# Autodesk Inventor assembly: assembly
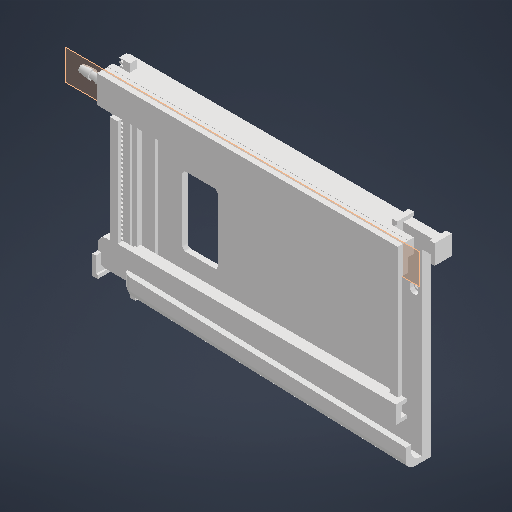
[picture p0: Inventor's stored thumbnail of the model, 512x512]
Saved by Autodesk Inventor 2026.2 (Build 302298010, 298A)
## iProperties
Created: 2026-07-05
Part Number: assembly
Document SubType Name: Assembly
Designer: pauli
Author: pauli
## Documents named in this file (6)
- D:\Documentos\auto-cleaning-solar-panel\hardware\CAD\iam\assembly.iam
- D:\Documentos\auto-cleaning-solar-panel\hardware\CAD\ipt\Gear.ipt
- D:\Documentos\auto-cleaning-solar-panel\hardware\CAD\ipt\Gear-Rack.ipt
- D:\Documentos\auto-cleaning-solar-panel\hardware\CAD\ipt\panel-suport.ipt
- D:\Documentos\auto-cleaning-solar-panel\hardware\CAD\ipt\Sprinkler.ipt
- D:\Documentos\auto-cleaning-solar-panel\hardware\CAD\ipt\Wiper-support.ipt
## Components (5 placed, 5 different names)
1. Gear:1 — Coincidente:7, Alinhado:1, Coincidente:8
2. Gear-Rack:1 — Coincidente:4, Coincidente:5, Coincidente:6, Coincidente:7, Alinhado:1, Coincidente:8
3. panel-suport:1 — Coincidente:1, Coincidente:2, Coincidente:3, Coincidente:4, Coincidente:5
4. Sprinkler:1 — Coincidente:1, Coincidente:2, Coincidente:3
5. Wiper-support:1 — Coincidente:6
## Relationships (9: Mate 8, Flush 1)
- Coincidente:1 [Mate]: panel-suport:1 ↔ Sprinkler:1
- Coincidente:2 [Mate]: panel-suport:1 ↔ Sprinkler:1
- Coincidente:3 [Mate]: panel-suport:1 ↔ Sprinkler:1
- Coincidente:4 [Mate]: Gear-Rack:1 ↔ panel-suport:1
- Coincidente:5 [Mate]: Gear-Rack:1 ↔ panel-suport:1
- Coincidente:6 [Mate]: Gear-Rack:1 ↔ Wiper-support:1
- Coincidente:7 [Mate]: Gear:1 ↔ Gear-Rack:1
- Alinhado:1 [Flush]: Gear:1 ↔ Gear-Rack:1
- Coincidente:8 [Mate]: Gear:1 ↔ Gear-Rack:1
